# Autodesk Inventor assembly: mmHexSocketHanger
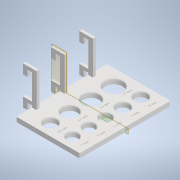
[picture p0: Inventor's stored thumbnail of the model, 180x180]
Saved by Autodesk Inventor 2020.3 (Build 243373000, 373)
## iProperties
Created: 2020-03-16
Part Number: mmHexSocketHanger
Document SubType Name: Assembly
Designer: robst
Author: robst
## Documents named in this file (3)
- C:\git\CAD-Development\robSteele\HouseProjects\Garage\Ikea\mmHexSocketHanger.iam
- C:\git\CAD-Development\robSteele\HouseProjects\Garage\Ikea\threeStartConfigurationV01.ipt
- C:\git\CAD-Development\robSteele\HouseProjects\Garage\Ikea\mmHexSocketSetOf9.ipt
## Components (2 placed, 2 different names)
1. threeStartConfigurationV01:1 — Mate:1, Flush:1, Flush:2
2. mmHexSocketSetOf9:1 — Mate:1, Flush:1, Flush:2
## Relationships (3: Flush 2, Mate 1)
- Mate:1: threeStartConfigurationV01:1 ↔ mmHexSocketSetOf9:1
- Flush:1: threeStartConfigurationV01:1 ↔ mmHexSocketSetOf9:1
- Flush:2: threeStartConfigurationV01:1 ↔ mmHexSocketSetOf9:1
